# Autodesk Inventor assembly: Car_Assembly
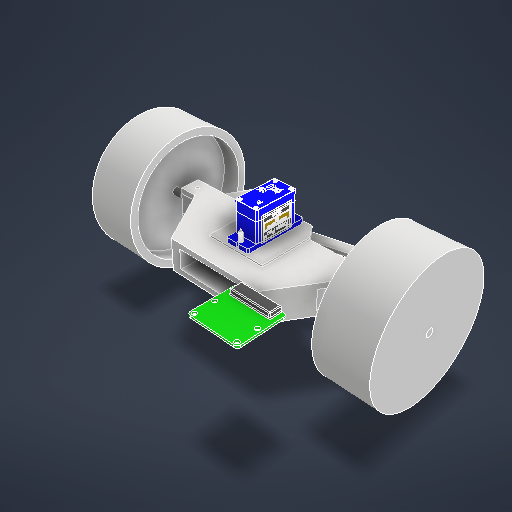
[picture p0: Inventor's stored thumbnail of the model, 512x512]
Saved by Autodesk Inventor 2025 (Build 290162000, 162)
## iProperties
Created: 2024-05-24
Part Number: Car_Assembly
Document SubType Name: Assembly
Designer: Garfieldcmix
Author: Garfieldcmix
## Documents named in this file (11)
- C:\Users\chaya\Desktop\WRO-2024-CAD\Car_Assembly.iam
- C:\Users\chaya\Desktop\WRO-2024-CAD\SG90 - Micro Servo 9g - Tower Pro\SG90 - Micro Servo 9g - Tower Pro.iam
- C:\Users\chaya\Desktop\WRO-2024-CAD\Front_Bridge.ipt
- C:\Users\chaya\Desktop\WRO-2024-CAD\SG90 - Micro Servo 9g - Tower Pro\SG90 - Micro Servo 9g - Tower Pro.2.ipt
- C:\Users\chaya\Desktop\WRO-2024-CAD\Front_Wheel_Anchor.ipt
- C:\Users\chaya\Desktop\WRO-2024-CAD\Front_Wheel_Anchor_MIR.ipt
- C:\Users\chaya\Desktop\WRO-2024-CAD\Wheel.ipt
- C:\Users\chaya\Desktop\WRO-2024-CAD\Wheel_MIR.ipt
- C:\Users\chaya\Desktop\WRO-2024-CAD\Servo_Steering_Linkage.ipt
- C:\Users\chaya\Desktop\WRO-2024-CAD\Servo_Steering_Linkage_MIR.ipt
- C:\Users\chaya\Desktop\WRO-2024-CAD\Pi camera module3\Pi camera module3.ipt
## Components (10 placed, 10 different names)
1. SG90_Servo [sub-assembly] — Mate:1, Mate:16, Mate:2, Mate:17
2. Servo_Arm — Mate:2, Mate:17, Mate:25, Mate:27, Mate:30, Mate:31
3. Front_Bridge:1 — Mate:1, Mate:16, Mate:18, Mate:19, Mate:21, Mate:22, Angle:1
4. Left_Front_Wheel_Anchor — Mate:18, Mate:19, Mate:20, Flush:1, Mate:24, Mate:26, Angle:1
5. Left_Front_Wheel — Mate:20, Flush:1
6. Right_Front_Wheel_Anchor — Mate:21, Mate:22, Mate:23, Flush:2, Mate:28, Mate:29
7. Right_Front_Wheel — Mate:23, Flush:2
8. Left_Servo_Steering_Linkage — Mate:24, Mate:25, Mate:26, Mate:27
9. Right_Servo_Steering_Linkage — Mate:28, Mate:31, Mate:29, Mate:30
10. Pi camera module3:1
## Relationships (21: Mate 18, Flush 2, Angle 1)
- Mate:1: SG90_Servo ↔ Front_Bridge:1
- Mate:16: SG90_Servo ↔ Front_Bridge:1
- Mate:2: SG90_Servo ↔ Servo_Arm
- Mate:17: SG90_Servo ↔ Servo_Arm
- Mate:18: Front_Bridge:1 ↔ Left_Front_Wheel_Anchor
- Mate:19: Front_Bridge:1 ↔ Left_Front_Wheel_Anchor
- Mate:20: Left_Front_Wheel_Anchor ↔ Left_Front_Wheel
- Flush:1: Left_Front_Wheel_Anchor ↔ Left_Front_Wheel
- Mate:21: Front_Bridge:1 ↔ Right_Front_Wheel_Anchor
- Mate:22: Front_Bridge:1 ↔ Right_Front_Wheel_Anchor
- Mate:23: Right_Front_Wheel_Anchor ↔ Right_Front_Wheel
- Flush:2: Right_Front_Wheel_Anchor ↔ Right_Front_Wheel
- Mate:24: Left_Front_Wheel_Anchor ↔ Left_Servo_Steering_Linkage
- Mate:25: Servo_Arm ↔ Left_Servo_Steering_Linkage
- Mate:26: Left_Front_Wheel_Anchor ↔ Left_Servo_Steering_Linkage
- Angle:1 (145 deg): Front_Bridge:1 ↔ Left_Front_Wheel_Anchor
- Mate:27: Servo_Arm ↔ Left_Servo_Steering_Linkage
- Mate:28: Right_Front_Wheel_Anchor ↔ Right_Servo_Steering_Linkage
- Mate:31: Servo_Arm ↔ Right_Servo_Steering_Linkage
- Mate:29: Right_Front_Wheel_Anchor ↔ Right_Servo_Steering_Linkage
- Mate:30: Servo_Arm ↔ Right_Servo_Steering_Linkage
